# Autodesk Inventor assembly: 110033226_iam_05_騎樓梁架_MIR
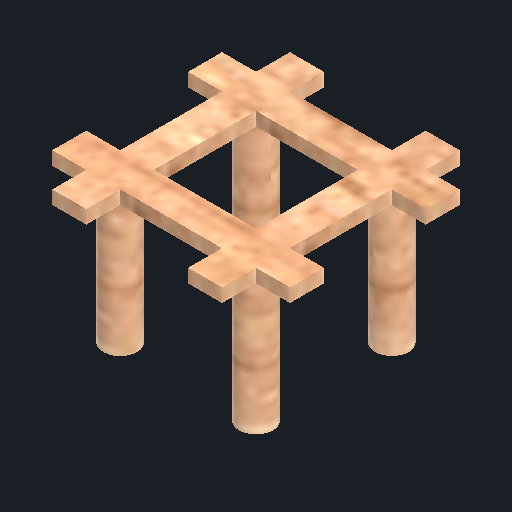
[picture p0: Inventor's stored thumbnail of the model, 512x512]
Saved by Autodesk Inventor 2022 (Build 260153000, 153)
## iProperties
Created: 2022-06-24
Part Number: 110033226_iam_05_騎樓梁架_MIR
Document SubType Name: Assembly
Designer: User
Author: User
## Documents named in this file (3)
- D:\D-disk\pomelo\大一\下學期\機械設計製圖\1100332260_LEGOproj_沒有公主城堡\110033226_iam_05_騎樓梁架_MIR.iam
- D:\D-disk\pomelo\大一\下學期\機械設計製圖\1100332260_LEGOproj_沒有公主城堡\110033226_ipt_27_騎樓梁架頂_MIR.ipt
- D:\D-disk\pomelo\大一\下學期\機械設計製圖\1100332260_LEGOproj_沒有公主城堡\110033226_ipt_26_騎樓梁架_MIR.ipt
## Components (2 placed, 2 different names)
1. 110033226_ipt_27_騎樓梁架頂_MIR:1 — 貼合:3, 貼合:2, 貼合:1
2. 110033226_ipt_26_騎樓梁架_MIR:1 — 貼合:3, 貼合:2, 貼合:1
## Relationships (3: Mate 3)
- 貼合:3 [Mate]: 110033226_ipt_27_騎樓梁架頂_MIR:1 ↔ 110033226_ipt_26_騎樓梁架_MIR:1
- 貼合:2 [Mate]: 110033226_ipt_27_騎樓梁架頂_MIR:1 ↔ 110033226_ipt_26_騎樓梁架_MIR:1
- 貼合:1 [Mate]: 110033226_ipt_27_騎樓梁架頂_MIR:1 ↔ 110033226_ipt_26_騎樓梁架_MIR:1
